# Autodesk Inventor assembly: 거치대 조립
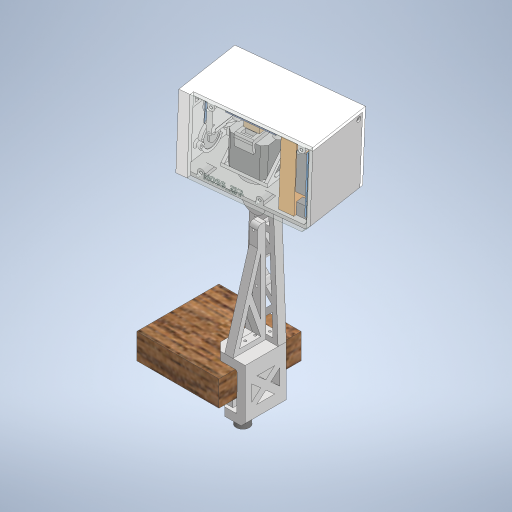
[picture p0: Inventor's stored thumbnail of the model, 512x512]
Saved by Autodesk Inventor 2023 (Build 270158000, 158)
## iProperties
Created: 2022-11-11
Part Number: 거치대 조립
Document SubType Name: Assembly
Designer: hyunsu
Author: hyunsu
## Documents named in this file (11)
- C:\Users\hyunsu\Desktop\동국대 메이커톤\설계\거치대\거치대 조립.iam
- C:\Users\hyunsu\Desktop\동국대 메이커톤\설계\거치대\나사 회전축.ipt
- C:\Users\hyunsu\Desktop\동국대 메이커톤\설계\거치대\메인 프레임.ipt
- C:\Users\hyunsu\Desktop\동국대 메이커톤\설계\거치대\보조 프레임.ipt
- C:\Users\hyunsu\Desktop\동국대 메이커톤\설계\거치대\책상 고정 판.ipt
- C:\Users\hyunsu\Desktop\동국대 메이커톤\설계\거치대\책상 고정판 홀더.ipt
- C:\Users\hyunsu\Desktop\동국대 메이커톤\설계\거치대\책상고정대.ipt
- C:\Users\hyunsu\Desktop\동국대 메이커톤\설계\제품 역설계\나사 10파이 30mm.ipt
- C:\Users\hyunsu\Desktop\동국대 메이커톤\설계\제품 역설계\테이블.ipt
- C:\Users\hyunsu\Desktop\동국대 메이커톤\설계\거치대\회전대.ipt
- C:\Users\hyunsu\Desktop\동국대 메이커톤\설계\NOSS조립.iam
## Components (10 placed, 10 different names)
1. 나사 회전축:1 — 삽입:2, 삽입:3
2. 메인 프레임:1 — 삽입:7, 삽입:8, 삽입:11, 각도:1
3. 보조 프레임:1 — 삽입:9, 삽입:10
4. 책상 고정 판:1 — 삽입:3, 플러쉬:2, 삽입:4
5. 책상 고정판 홀더:1 — 삽입:4
6. 책상고정대:1 — 메이트:1, 메이트:2, 플러쉬:1, 삽입:1, 플러쉬:2, 삽입:7, 삽입:8, 삽입:9, 삽입:10
7. 나사 10파이 30mm:1 — 삽입:1, 삽입:2
8. 테이블:1 — 메이트:1, 메이트:2, 플러쉬:1
9. 회전대:1 — 삽입:11, 각도:1, 삽입:12
10. NOSS조립:1 [sub-assembly] — 삽입:12
## Relationships (15: Insert 10, Mate 2, Flush 2, Angle 1)
- 메이트:1 [Mate]: 책상고정대:1 ↔ 테이블:1
- 메이트:2 [Mate] (2 mm): 책상고정대:1 ↔ 테이블:1
- 플러쉬:1 [Flush] (-20 mm): 책상고정대:1 ↔ 테이블:1
- 삽입:1 [Insert] (12 mm): 책상고정대:1 ↔ 나사 10파이 30mm:1
- 삽입:2 [Insert]: 나사 회전축:1 ↔ 나사 10파이 30mm:1
- 삽입:3 [Insert]: 나사 회전축:1 ↔ 책상 고정 판:1
- 플러쉬:2 [Flush]: 책상 고정 판:1 ↔ 책상고정대:1
- 삽입:4 [Insert]: 책상 고정 판:1 ↔ 책상 고정판 홀더:1
- 삽입:7 [Insert]: 메인 프레임:1 ↔ 책상고정대:1
- 삽입:8 [Insert]: 메인 프레임:1 ↔ 책상고정대:1
- 삽입:9 [Insert]: 보조 프레임:1 ↔ 책상고정대:1
- 삽입:10 [Insert]: 보조 프레임:1 ↔ 책상고정대:1
- 삽입:11 [Insert]: 메인 프레임:1 ↔ 회전대:1
- 각도:1 [Angle] (0 deg): 메인 프레임:1 ↔ 회전대:1
- 삽입:12 [Insert]: 회전대:1 ↔ NOSS조립:1
